# Autodesk Inventor assembly: 1-Post Hex Nut Retainer With Hardware
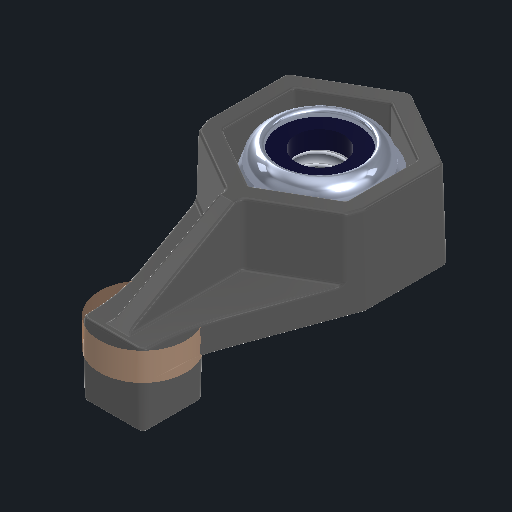
[picture p0: Inventor's stored thumbnail of the model, 512x512]
Saved by Autodesk Inventor 2025 (Build 290162000, 162)
## iProperties
Created: 2024-11-07
Part Number: 1-Post Hex Nut Retainer With Hardware
Document SubType Name: Assembly
Designer: avere
Author: avere
## Documents named in this file (3)
- D:\VEX\High Stakes\CAD\ROBOPROS-CAD-Inventor\Structure\1-Post Hex Nut Retainer With Hardware.iam
- D:\VEX\High Stakes\CAD\ROBOPROS-CAD-Inventor\Structure\1-Post Hex Nut Retainer.ipt
- D:\VEX\High Stakes\CAD\ROBOPROS-CAD-Inventor\Structure\Hardware\Nut Thin Nylock.ipt
## Components (2 placed, 2 different names)
1. 1-Post Hex Nut Retainer:1 — Insert:1
2. Nut Thin Nylock:1 — Insert:1
## Relationships (1: Insert 1)
- Insert:1: 1-Post Hex Nut Retainer:1 ↔ Nut Thin Nylock:1
